# Autodesk Inventor assembly: 足 前サスギア アセンブリ
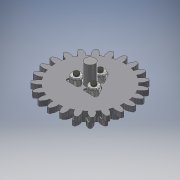
[picture p0: Inventor's stored thumbnail of the model, 180x180]
Saved by Autodesk Inventor 2016 (Build 200138000, 138)
## iProperties
Created: 2019-10-21
Part Number: 足 前サスギア アセンブリ
Material: 一般
Document SubType Name: Assembly
Designer: mozar
Author: mozar
## Documents named in this file (7)
- C:\Users\mozar\Desktop\院2年機\既製品\ねじ\足 前サスギア アセンブリ.iam
- C:\Users\mozar\Desktop\院2年機\足 前サス軸大ギア.ipt
- C:\Users\mozar\Desktop\院2年機\足 前サス軸ギア繋ぎカム.ipt
- C:\Users\mozar\Desktop\院2年機\足 前サス軸小ギア.ipt
- C:\Users\mozar\Desktop\院2年機\既製品\ねじ\ナイロンナットm3.ipt
- C:\Users\mozar\Desktop\院2年機\既製品\ねじ\SB　18mm皿ネジ.ipt
- C:\Users\mozar\Desktop\院2年機\既製品\平行ピン　φ6　長さ30.ipt
## Components (10 placed, 6 different names)
1. 足 前サス軸大ギア:1 — 挿入:1, 挿入:2, 挿入:5, 挿入:6, 挿入:7, メイト:1, メイト:2, メイト:3
2. 足 前サス軸ギア繋ぎカム:1 — 挿入:1, 挿入:2, 挿入:3, 挿入:4
3. 足 前サス軸小ギア:1 — 挿入:3, 挿入:4, 挿入:8, 挿入:9, 挿入:10, 挿入:11
4. ナイロンナットm3:1 — 挿入:5, メイト:1
5. ナイロンナットm3:2 — 挿入:6, メイト:2
6. ナイロンナットm3:3 — 挿入:7, メイト:3
7. SB　18mm皿ネジ:1 — 挿入:10
8. SB　18mm皿ネジ:2 — 挿入:9
9. SB　18mm皿ネジ:3 — 挿入:8
10. 平行ピン　φ6　長さ30:1 — 挿入:11
## Relationships (14: Insert 11, Mate 3)
- 挿入:1 [Insert]: 足 前サス軸大ギア:1 ↔ 足 前サス軸ギア繋ぎカム:1
- 挿入:2 [Insert]: 足 前サス軸大ギア:1 ↔ 足 前サス軸ギア繋ぎカム:1
- 挿入:3 [Insert]: 足 前サス軸ギア繋ぎカム:1 ↔ 足 前サス軸小ギア:1
- 挿入:4 [Insert]: 足 前サス軸ギア繋ぎカム:1 ↔ 足 前サス軸小ギア:1
- 挿入:5 [Insert]: 足 前サス軸大ギア:1 ↔ ナイロンナットm3:1
- 挿入:6 [Insert]: 足 前サス軸大ギア:1 ↔ ナイロンナットm3:2
- 挿入:7 [Insert]: 足 前サス軸大ギア:1 ↔ ナイロンナットm3:3
- メイト:1 [Mate]: 足 前サス軸大ギア:1 ↔ ナイロンナットm3:1
- メイト:2 [Mate]: 足 前サス軸大ギア:1 ↔ ナイロンナットm3:2
- メイト:3 [Mate]: 足 前サス軸大ギア:1 ↔ ナイロンナットm3:3
- 挿入:8 [Insert]: 足 前サス軸小ギア:1 ↔ SB　18mm皿ネジ:3
- 挿入:9 [Insert]: 足 前サス軸小ギア:1 ↔ SB　18mm皿ネジ:2
- 挿入:10 [Insert]: 足 前サス軸小ギア:1 ↔ SB　18mm皿ネジ:1
- 挿入:11 [Insert] (-5 mm): 足 前サス軸小ギア:1 ↔ 平行ピン　φ6　長さ30:1
